# Autodesk Inventor assembly: nc_nhk22
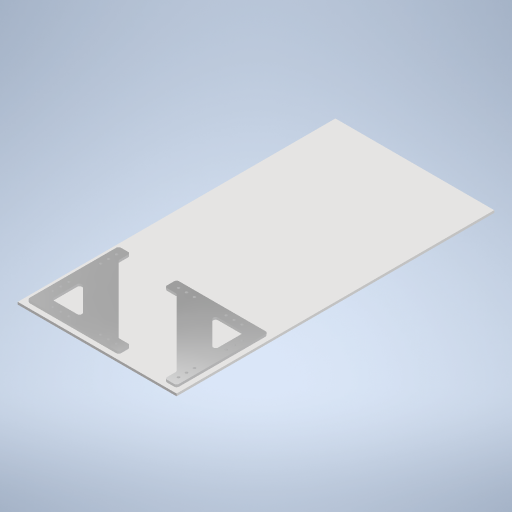
[picture p0: Inventor's stored thumbnail of the model, 512x512]
Saved by Autodesk Inventor 2023 (Build 270158000, 158)
## iProperties
Created: 2022-04-30
Part Number: nc_nhk22
Document SubType Name: Assembly
Designer: yuta
Author: yuta
## Documents named in this file (3)
- C:\Users\yuta\Documents\NHK\nc_nhk22.iam
- C:\Users\yuta\Documents\NHK\NC.port.ipt
- C:\Users\yuta\Documents\NHK\射出_固定2.ipt
## Components (3 placed, 2 different names)
1. NC.port:1 — メイト:1, フラッシュ:1, フラッシュ:2, メイト:2, フラッシュ:3, フラッシュ:4
2. 射出_固定2:1 — メイト:2, フラッシュ:3, フラッシュ:4
3. 射出_固定2:2 — メイト:1, フラッシュ:1, フラッシュ:2
## Relationships (6: Flush 4, Mate 2)
- メイト:1 [Mate]: NC.port:1 ↔ 射出_固定2:2
- フラッシュ:1 [Flush] (6 mm): NC.port:1 ↔ 射出_固定2:2
- フラッシュ:2 [Flush] (6 mm): NC.port:1 ↔ 射出_固定2:2
- メイト:2 [Mate]: NC.port:1 ↔ 射出_固定2:1
- フラッシュ:3 [Flush] (6 mm): NC.port:1 ↔ 射出_固定2:1
- フラッシュ:4 [Flush] (6 mm): NC.port:1 ↔ 射出_固定2:1
